# Autodesk Inventor assembly: Base_Plate_Assembly
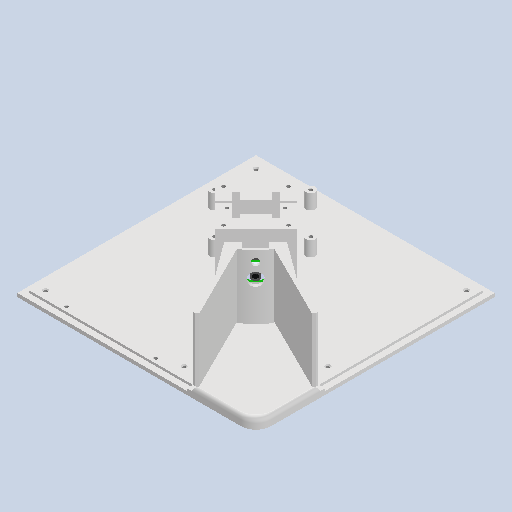
[picture p0: Inventor's stored thumbnail of the model, 512x512]
Saved by Autodesk Inventor 2022 (Build 260153000, 153)
## iProperties
Created: 2023-02-28
Part Number: Base_Plate_Assembly
Document SubType Name: Assembly
Designer: zarek
Author: zarek
## Documents named in this file (5)
- C:\Users\zarek\OneDrive\Desktop\Random New Stuff\SPB\Base_Plate_Assembly.iam
- C:\Users\zarek\OneDrive\Desktop\Random New Stuff\SPB\GrabCad Parts\Pi camera module3 (1).ipt
- C:\Users\zarek\OneDrive\Desktop\Random New Stuff\SPB\Motor_Holder.ipt
- C:\Users\zarek\OneDrive\Desktop\Random New Stuff\SPB\Base_Plate_2_Solo.ipt
- C:\Users\zarek\OneDrive\Desktop\Random New Stuff\SPB\Camera_Holder.ipt
## Components (4 placed, 4 different names)
1. Motor_Holder:1 — Rigid:1
2. Base_Plate_2_Solo:1 — Rigid:1, Mate:1
3. Pi camera module3 (1):1 — Rotational:1
4. Camera_Holder:1 — Mate:1, Rotational:1
## Relationships (3: WeldJoint 1, Mate 1, RevoluteJoint 1)
- Rigid:1 [WeldJoint]: Motor_Holder:1 ↔ Base_Plate_2_Solo:1
- Mate:1: Base_Plate_2_Solo:1 ↔ Camera_Holder:1
- Rotational:1 [RevoluteJoint]: Pi camera module3 (1):1 ↔ Camera_Holder:1
